# Autodesk Inventor assembly: Universal Joint
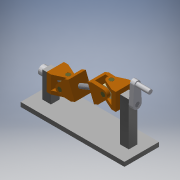
[picture p0: Inventor's stored thumbnail of the model, 180x180]
Saved by Autodesk Inventor 2019 Beta2 (Build 230110000, 110) ContinuousBuild 0
## iProperties
Created: 2014-03-04
Part Number: Universal Joint
Document SubType Name: Assembly
Designer: John
Author: John
## Documents named in this file (8)
- C:\Users\helfenj\Desktop\Ex_Files_Autodesk_Inventor_2019_EssT\Exercise Files\13_Adding parts to an assembly file\13_01\Universal Joint.iam
- C:\Users\helfenj\Desktop\Ex_Files_Autodesk_Inventor_2019_EssT\Exercise Files\13_Adding parts to an assembly file\13_01\base.ipt
- C:\Users\helfenj\Desktop\Ex_Files_Autodesk_Inventor_2019_EssT\Exercise Files\13_Adding parts to an assembly file\13_01\Connector.ipt
- C:\Users\helfenj\Desktop\Ex_Files_Autodesk_Inventor_2019_EssT\Exercise Files\13_Adding parts to an assembly file\13_01\Joint.ipt
- C:\Users\helfenj\Desktop\Ex_Files_Autodesk_Inventor_2019_EssT\Exercise Files\13_Adding parts to an assembly file\13_01\Connecting Rod.ipt
- C:\Users\helfenj\Desktop\Ex_Files_Autodesk_Inventor_2019_EssT\Exercise Files\13_Adding parts to an assembly file\13_01\Crank Rod.ipt
- C:\Users\helfenj\Desktop\Ex_Files_Autodesk_Inventor_2019_EssT\Exercise Files\13_Adding parts to an assembly file\13_01\Crank Handle.ipt
- C:\Users\helfenj\Desktop\Ex_Files_Autodesk_Inventor_2019_EssT\Exercise Files\13_Adding parts to an assembly file\13_01\Pin.ipt
## Components (20 placed, 8 different names)
1. base:1 — Mate:1, Mate:2, Mate:9, Mate:10, Mate:15, Mate:16, Angle:3 - DRIVE THIS
2. Connector:1 — Mate:3, Mate:4, Mate:7, Mate:8
3. Connector:2 — Mate:5, Mate:6, Mate:11, Mate:12
4. Joint:1 — Mate:1, Mate:2, Mate:3, Mate:4, Flush:3, Angle:1, Insert:1, Insert:2
5. Joint:2 — Mate:5, Mate:6, Mate:9, Mate:10, Flush:4, Angle:2, Insert:5, Insert:8
6. Joint:3 — Mate:7, Mate:8, Mate:13, Flush:1, Mate:14, Insert:3, Insert:4
7. Joint:4 — Mate:11, Mate:12, Mate:13, Flush:1, Flush:2, Insert:6, Insert:7
8. Connecting Rod:1 — Mate:14, Flush:2
9. Crank Rod:1 — Mate:15, Flush:3, Flush:5, Mate:17
10. Crank Rod:2 — Flush:4, Mate:16, Flush:6, Mate:18
11. Crank Handle:1 - DRIVE — Flush:5, Mate:17, Angle:1, Angle:3 - DRIVE THIS
12. Crank Handle:2 — Flush:6, Angle:2, Mate:18
13. Pin:1 — Insert:1
14. Pin:2 — Insert:4
15. Pin:3 — Insert:3
16. Pin:4 — Insert:2
17. Pin:5 — Insert:7
18. Pin:6 — Insert:8
19. Pin:7 — Insert:6
20. Pin:8 — Insert:5
## Relationships (35: Mate 18, Insert 8, Flush 6, Angle 3)
- Mate:1: base:1 ↔ Joint:1
- Mate:2: base:1 ↔ Joint:1
- Mate:3: Connector:1 ↔ Joint:1
- Mate:4 (1.27 mm): Connector:1 ↔ Joint:1
- Mate:5: Connector:2 ↔ Joint:2
- Mate:6 (1.27 mm): Connector:2 ↔ Joint:2
- Mate:7: Connector:1 ↔ Joint:3
- Mate:8 (1.27 mm): Connector:1 ↔ Joint:3
- Mate:9: base:1 ↔ Joint:2
- Mate:10: base:1 ↔ Joint:2
- Mate:11: Connector:2 ↔ Joint:4
- Mate:12 (1.27 mm): Connector:2 ↔ Joint:4
- Mate:13: Joint:3 ↔ Joint:4
- Flush:1: Joint:3 ↔ Joint:4
- Mate:14: Joint:3 ↔ Connecting Rod:1
- Flush:2: Joint:4 ↔ Connecting Rod:1
- Mate:15: base:1 ↔ Crank Rod:1
- Flush:3: Joint:1 ↔ Crank Rod:1
- Flush:4: Joint:2 ↔ Crank Rod:2
- Mate:16: base:1 ↔ Crank Rod:2
- Flush:5: Crank Rod:1 ↔ Crank Handle:1 - DRIVE
- Mate:17: Crank Rod:1 ↔ Crank Handle:1 - DRIVE
- Angle:1 (0 deg): Joint:1 ↔ Crank Handle:1 - DRIVE
- Flush:6: Crank Rod:2 ↔ Crank Handle:2
- Angle:2 (45 deg): Joint:2 ↔ Crank Handle:2
- Mate:18: Crank Rod:2 ↔ Crank Handle:2
- Insert:1: Joint:1 ↔ Pin:1
- Insert:2: Joint:1 ↔ Pin:4
- Insert:3: Joint:3 ↔ Pin:3
- Insert:4: Joint:3 ↔ Pin:2
- Insert:5: Joint:2 ↔ Pin:8
- Insert:6: Joint:4 ↔ Pin:7
- Insert:7: Joint:4 ↔ Pin:5
- Insert:8: Joint:2 ↔ Pin:6
- Angle:3 - DRIVE THIS (180 deg): base:1 ↔ Crank Handle:1 - DRIVE
